# Autodesk Inventor assembly: McCrea_final_scene_walle
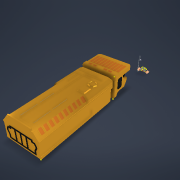
[picture p0: Inventor's stored thumbnail of the model, 180x180]
Saved by Autodesk Inventor 2022 (Build 260153000, 153)
## iProperties
Created: 2022-02-01
Part Number: McCrea_final_scene_walle
Document SubType Name: Assembly
Designer: MatusBarany
Author: MatusBarany
## Documents named in this file (6)
- C:\Users\MatusBarany\Documents\Inventor\wall-e\assembly\McCrea_final_scene_walle.iam
- C:\Users\MatusBarany\Documents\Inventor\wall-e\matus\bench\McCrea_assembly_walle.iam
- C:\Users\MatusBarany\Documents\Inventor\wall-e\assembly\McCrea_WALLE_bez_HEAD_walle.iam
- C:\Users\MatusBarany\Documents\Inventor\wall-e\matus\lampa\McCrea_lampa_walle.ipt
- C:\Users\MatusBarany\Documents\Inventor\wall-e\matus\electronic truck\McCrea_roof_walle.ipt
- C:\Users\MatusBarany\Documents\Inventor\wall-e\lukas\McCrea_Auto_walle.ipt
## Components (5 placed, 5 different names)
1. McCrea_assembly_walle:1 [sub-assembly]
2. McCrea_WALLE_bez_HEAD_walle:1 [sub-assembly]
3. McCrea_lampa_walle:1
4. McCrea_roof_walle:1 — Flush:1
5. McCrea_Auto_walle:1 — Flush:1
## Relationships (1: Flush 1)
- Flush:1: McCrea_roof_walle:1 ↔ McCrea_Auto_walle:1
